# Autodesk Inventor assembly: Power
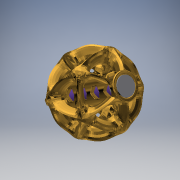
[picture p0: Inventor's stored thumbnail of the model, 180x180]
Saved by Autodesk Inventor 2019 (Build 230136000, 136)
## iProperties
Created: 2019-05-09
Part Number: Power
Document SubType Name: Assembly
Designer: Jorian Brusind
Author: Jorian Brusind
## Documents named in this file (4)
- C:\Users\Jorian Brusind\Documents\GitHub\PersonalProjects\Inventor Projects\Infinity\Power.iam
- C:\Users\Jorian Brusind\Documents\GitHub\PersonalProjects\Inventor Projects\Infinity\Purple.ipt
- C:\Users\Jorian Brusind\Documents\GitHub\PersonalProjects\Inventor Projects\Infinity\Orb.ipt
- C:\Users\Jorian Brusind\Documents\GitHub\PersonalProjects\Inventor Projects\Infinity\EndCap.ipt
## Components (4 placed, 3 different names)
1. Purple:1 — Mate:1, Mate:6
2. Orb:1 — Mate:1, Mate:3, Mate:4, Mate:5, Flush:1
3. EndCap:1 — Mate:3, Flush:1, Mate:6
4. EndCap:2 — Mate:4, Mate:5
## Relationships (6: Mate 5, Flush 1)
- Mate:1: Purple:1 ↔ Orb:1
- Mate:3: Orb:1 ↔ EndCap:1
- Mate:4: Orb:1 ↔ EndCap:2
- Mate:5: Orb:1 ↔ EndCap:2
- Flush:1: Orb:1 ↔ EndCap:1
- Mate:6: Purple:1 ↔ EndCap:1
## Named parameters: sa_0 = 6894.76
note: some values were not read from the file. Shown as the stored number, unit unknown: "sa_0".
